# Autodesk Inventor assembly: pulley
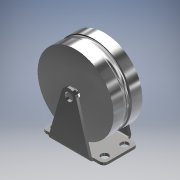
[picture p0: Inventor's stored thumbnail of the model, 180x180]
Saved by Autodesk Inventor 2018 (Build 220112000, 112)
## iProperties
Created: 2018-11-15
Part Number: pulley
Document SubType Name: Assembly
Designer: Admin
Author: Admin
## Documents named in this file (3)
- C:\Users\Admin\Documents\Cryostat\CAD\pulley.iam
- C:\Users\Admin\Documents\Cryostat\CAD\pulley wheel.ipt
- C:\Users\Admin\Documents\Cryostat\CAD\pulley holder.ipt
## Components (2 placed, 2 different names)
1. pulley wheel:1 — Mate:1, Mate:2
2. pulley holder:1 — Mate:1, Mate:2
## Relationships (2: Mate 2)
- Mate:1: pulley wheel:1 ↔ pulley holder:1
- Mate:2 (2.9972 mm): pulley wheel:1 ↔ pulley holder:1
